# Autodesk Inventor assembly: Trebuchet Assembly
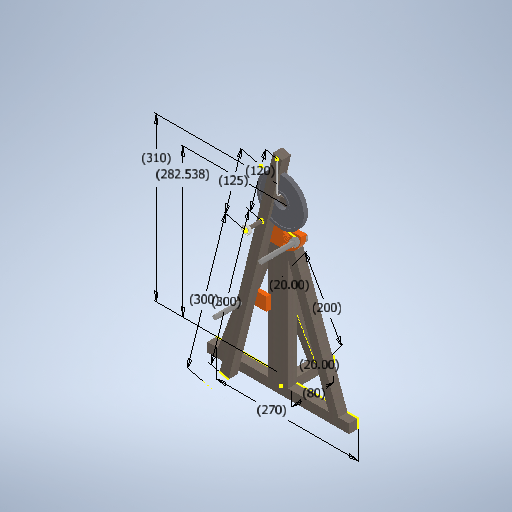
[picture p0: Inventor's stored thumbnail of the model, 512x512]
Saved by Autodesk Inventor 2025.2 (Build 292293000, 293)
## iProperties
Created: 2025-02-17
Part Number: Trebuchet Assembly
Document SubType Name: Assembly
Designer: baolo
Mass: 1433.08 g
Surface Area: 3943.53 cm^2
Volume: 1805.19 cm^3
Density: 0.793867 g/cm^3
Author: baolo
## Documents named in this file (9)
- C:\Users\baolo\OneDrive\Desktop\the 2024 homework folder\engg 160\Trebuchet Models\Trebuchet Assembly.iam
- C:\Users\baolo\OneDrive\Desktop\the 2024 homework folder\engg 160\Trebuchet Models\Long Arm.ipt
- C:\Users\baolo\OneDrive\Desktop\the 2024 homework folder\engg 160\Trebuchet Models\Counterweight (500g).ipt
- C:\Users\baolo\OneDrive\Desktop\the 2024 homework folder\engg 160\Trebuchet Models\Mock String.ipt
- C:\Users\baolo\OneDrive\Desktop\the 2024 homework folder\engg 160\Trebuchet Models\Jet Base Design.iam
- C:\Users\baolo\OneDrive\Desktop\the 2024 homework folder\engg 160\Trebuchet Models\60355K151_Ball Bearing\60355K151_Ball Bearing\60355K151_Ball Bearing.ipt
- C:\Users\baolo\OneDrive\Desktop\the 2024 homework folder\engg 160\Trebuchet Models\AnglePlate.iam
- C:\Users\baolo\OneDrive\Desktop\the 2024 homework folder\engg 160\Trebuchet Models\BoltRelease.ipt
- C:\Users\baolo\OneDrive\Documents\Inventor\Content Center Files\R2025\en-US\BS EN ISO 4017\BS EN ISO 4017 - M8 x 80BS EN.ipt
## Components (10 placed, 8 different names)
1. Long Arm:1 — Mate:15, Insert:1, Insert:2, Tangent:10, Flush:14, Mate:18
2. Counterweight (500g):1 — Mate:10, Tangent:3, Tangent:5, Tangent:8, Mate:18
3. Mock String:1 — Angle:1, Mate:10, Tangent:5, Tangent:7, Tangent:9, Tangent:10
4. Jet Base Design:1 [sub-assembly] — Mate:12, Flush:10, Mate:13, Symmetry:1, Mate:15
5. Jet Base Design:2 [sub-assembly] — Mate:11, Flush:10, Mate:13, Symmetry:1, Flush:11, Mate:16, Flush:12, Flush:13, Mate:17
6. 60355K151_Ball Bearing:1 — Insert:1
7. 60355K151_Ball Bearing:2 — Insert:2
8. AnglePlate:1 [sub-assembly] — Mate:16, Flush:12, Flush:13
9. BoltRelease:1 — Mate:17, Insert:3
10. BS EN ISO 4017 - Metric M8 x 80:1 — Insert:3
## Relationships (27: Mate 10, Tangent 6, Flush 5, Insert 3, Angle 2, Symmetry 1)
- Mate:4
- Angle:1 (180 deg): Mock String:1
- Mate:10: Counterweight (500g):1 ↔ Mock String:1
- Mate:11: Jet Base Design:2
- Mate:12: Jet Base Design:1
- Flush:10: Jet Base Design:1 ↔ Jet Base Design:2
- Mate:13 (45 mm): Jet Base Design:1 ↔ Jet Base Design:2
- Symmetry:1: Jet Base Design:1 ↔ Jet Base Design:2
- Mate:14
- Mate:15: Long Arm:1 ↔ Jet Base Design:1
- Flush:11: Jet Base Design:2
- Tangent:3: Counterweight (500g):1
- Tangent:5: Counterweight (500g):1 ↔ Mock String:1
- Tangent:7: Mock String:1
- Angle:4 (0 deg)
- Tangent:8: Counterweight (500g):1
- Tangent:9: Mock String:1
- Insert:1: Long Arm:1 ↔ 60355K151_Ball Bearing:1
- Insert:2: Long Arm:1 ↔ 60355K151_Ball Bearing:2
- Mate:16: Jet Base Design:2 ↔ AnglePlate:1
- Flush:12: Jet Base Design:2 ↔ AnglePlate:1
- Flush:13 (39.8 mm): Jet Base Design:2 ↔ AnglePlate:1
- Tangent:10: Long Arm:1 ↔ Mock String:1
- Mate:17: Jet Base Design:2 ↔ BoltRelease:1
- Flush:14: Long Arm:1
- Insert:3: BoltRelease:1 ↔ BS EN ISO 4017 - Metric M8 x 80:1
- Mate:18: Long Arm:1 ↔ Counterweight (500g):1
## Named parameters: test = 1 mm
